# Autodesk Inventor assembly: 14
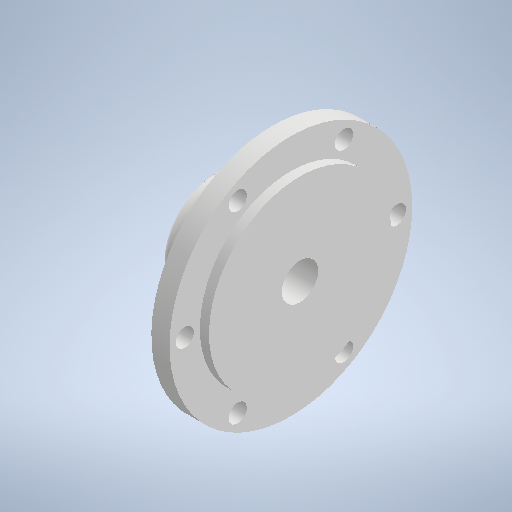
[picture p0: Inventor's stored thumbnail of the model, 512x512]
Saved by Autodesk Inventor 2025.1 (Build 291241000, 241)
## iProperties
Created: 2024-09-13
Part Number: 14
Document SubType Name: Assembly
Designer: ffogue
Author: ffogue
## Documents named in this file (3)
- C:\Users\ffogue\Documents\Inventor\Single cylinder Steam Engine\14.iam
- C:\Users\ffogue\Documents\Inventor\Single cylinder Steam Engine\14.ipt
- C:\Users\ffogue\Documents\Inventor\Single cylinder Steam Engine\14.2.ipt
## Components (2 placed, 2 different names)
1. 14:1 — Mate:1, Insert:1
2. 14.2:1 — Mate:1, Insert:1
## Relationships (2: Mate 1, Insert 1)
- Mate:1: 14:1 ↔ 14.2:1
- Insert:1: 14:1 ↔ 14.2:1
